# Autodesk Inventor assembly: Assembly
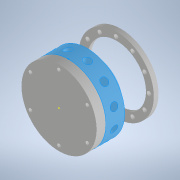
[picture p0: Inventor's stored thumbnail of the model, 180x180]
Saved by Autodesk Inventor 2021 (Build 250183000, 183)
## iProperties
Created: 2022-11-15
Part Number: Assembly
Document SubType Name: Assembly
Designer: warre
Author: warre
## Documents named in this file (5)
- D:\VUB\MA1\MA1 project\Assembly.iam
- D:\VUB\MA1\MA1 project\diaphragm.ipt
- D:\VUB\MA1\MA1 project\inner tube.ipt
- D:\VUB\MA1\MA1 project\magnet bottom.ipt
- D:\VUB\MA1\MA1 project\top ring.ipt
## Components (4 placed, 4 different names)
1. diaphragm:1 — Rigid:1, Cylindrical:1, Mate:1
2. inner tube:1 — Mate:1
3. magnet bottom:1 — Rigid:1
4. top ring:1 — Cylindrical:1
## Relationships (3: WeldJoint 1, CylindricalJoint 1, Mate 1)
- Rigid:1 [WeldJoint] (-10 mm): diaphragm:1 ↔ magnet bottom:1
- Cylindrical:1: diaphragm:1 ↔ top ring:1
- Mate:1: diaphragm:1 ↔ inner tube:1
